# Autodesk Inventor assembly: 25_Truc_dan
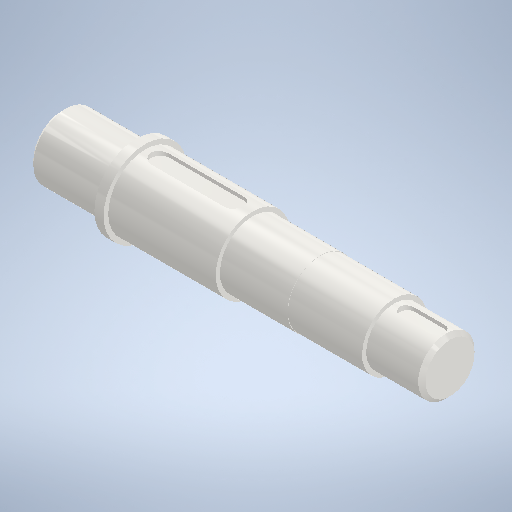
[picture p0: Inventor's stored thumbnail of the model, 512x512]
Saved by Autodesk Inventor 2025.2 (Build 292293000, 293)
## iProperties
Created: 2024-11-26
Part Number: 25_Truc_dan
Document SubType Name: Assembly
Designer: hongquan
Author: hongquan
## Documents named in this file (2)
- C:\Users\hongquan\Documents\GitHub\Optimal-Design-Robot\Inventor\Hopgiamtoc\25_Truc_dan.iam
- C:\Users\hongquan\Documents\GitHub\Optimal-Design-Robot\Inventor\Hopgiamtoc\Shaft1.ipt
## Components (1 placed, 1 different names)
1. Shaft:1 — Tangent:1, Tangent:2
## Relationships (4: Angle 2, Tangent 2)
- Angle:1 (0 deg)
- Tangent:1: Shaft:1
- Angle:2 (0 deg)
- Tangent:2: Shaft:1
